# Autodesk Inventor assembly: Rover Swerve Drive Mount 1.19
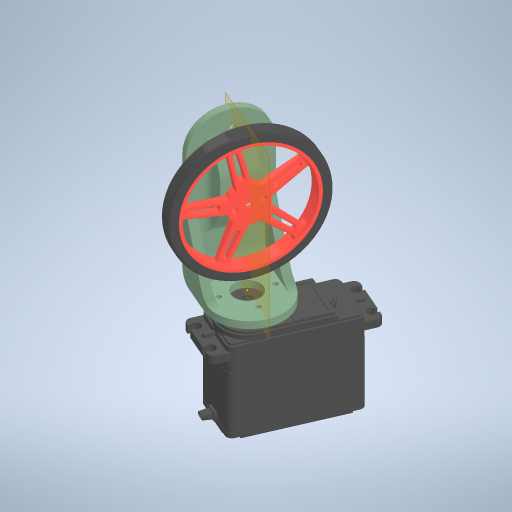
[picture p0: Inventor's stored thumbnail of the model, 512x512]
Saved by Autodesk Inventor 2024 (Build 280153000, 153)
## iProperties
Created: 2024-01-13
Part Number: Rover Swerve Drive Mount 1.19
Document SubType Name: Assembly
Designer: student
Author: student
## Documents named in this file (8)
- E:\TRACER DOCUMENTS\SheetMetal\Rover Swerve Drive Mount 1.19.iam
- E:\TRACER DOCUMENTS\SheetMetal\Servo 775 (with Spline).iam
- E:\TRACER DOCUMENTS\Swerve Drive\dcmotorLBracklet.ipt
- E:\TRACER DOCUMENTS\SheetMetal\N20Motor.iam
- E:\TRACER DOCUMENTS\SheetMetal\RedWheel.ipt
- E:\TRACER DOCUMENTS\SheetMetal\motorholder bracket 2.0.ipt
- E:\TRACER DOCUMENTS\SheetMetal\N20Bracklet- Left.ipt
- E:\TRACER DOCUMENTS\SheetMetal\N20Bracklet-Holder.ipt
## Components (7 placed, 7 different names)
1. Servo 775 (with Spline):1 [sub-assembly] — Flush:1, Mate:2, Angle:1
2. dcmotorLBracklet:1 — Flush:1, Mate:2, Angle:1, Angle:2, Mate:7, Mate:8, Mate:9, Flush:2, Mate:12
3. N20Motor:1 [sub-assembly] — Angle:2, Mate:7, Mate:8, Mate:10, Mate:11, Flush:3
4. motorholder bracket 2.0:1 — Flush:2
5. RedWheel:1 — Mate:9, Mate:10
6. N20Bracklet- Left:1 — Mate:11, Mate:12, Flush:3, Flush:4
7. N20Bracklet-Holder:1 — Flush:4
## Relationships (13: Mate 7, Flush 4, Angle 2)
- Flush:1: Servo 775 (with Spline):1 ↔ dcmotorLBracklet:1
- Mate:2: Servo 775 (with Spline):1 ↔ dcmotorLBracklet:1
- Angle:1 (0 deg): Servo 775 (with Spline):1 ↔ dcmotorLBracklet:1
- Angle:2 (0 deg): dcmotorLBracklet:1 ↔ N20Motor:1
- Mate:7: dcmotorLBracklet:1 ↔ N20Motor:1
- Mate:8: dcmotorLBracklet:1 ↔ N20Motor:1
- Mate:9: dcmotorLBracklet:1 ↔ RedWheel:1
- Mate:10: N20Motor:1 ↔ RedWheel:1
- Flush:2: dcmotorLBracklet:1 ↔ motorholder bracket 2.0:1
- Mate:11: N20Motor:1 ↔ N20Bracklet- Left:1
- Mate:12: dcmotorLBracklet:1 ↔ N20Bracklet- Left:1
- Flush:3: N20Motor:1 ↔ N20Bracklet- Left:1
- Flush:4: N20Bracklet- Left:1 ↔ N20Bracklet-Holder:1
